# Autodesk Inventor assembly: MM3_3
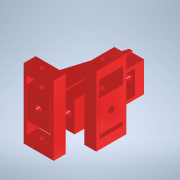
[picture p0: Inventor's stored thumbnail of the model, 180x180]
Saved by Autodesk Inventor 2021 (Build 250183000, 183)
## iProperties
Created: 2021-02-23
Part Number: MM3_3
Document SubType Name: Assembly
Designer: dsdan
Author: dsdan
## Documents named in this file (3)
- E:\OneDrive - Imperial College London\DragonVision_DanielKo\Instrumentation\Ephys_rig_2021\MM3_3.iam
- E:\OneDrive - Imperial College London\DragonVision_DanielKo\Instrumentation\Ephys_rig_2021\MM3.iam
- E:\OneDrive - Imperial College London\DragonVision_DanielKo\Instrumentation\Ephys_rig_2021\MM3_vertical.ipt
## Components (4 placed, 2 different names)
1. MM3:1 [sub-assembly] — Mate:1, Mate:2, Flush:1, Mate:4, Angle:1
2. MM3_vertical:1 — Mate:1, Mate:2, Flush:1, Mate:3, Flush:2
3. MM3:3 [sub-assembly] — Mate:3, Flush:2, Mate:4, Mate:5, Mate:6
4. MM3:4 [sub-assembly] — Mate:5, Angle:1, Mate:6
## Relationships (9: Mate 6, Flush 2, Angle 1)
- Mate:1: MM3:1 ↔ MM3_vertical:1
- Mate:2: MM3:1 ↔ MM3_vertical:1
- Flush:1: MM3:1 ↔ MM3_vertical:1
- Mate:3: MM3_vertical:1 ↔ MM3:3
- Flush:2: MM3_vertical:1 ↔ MM3:3
- Mate:4: MM3:1 ↔ MM3:3
- Mate:5: MM3:3 ↔ MM3:4
- Angle:1 (0 deg): MM3:1 ↔ MM3:4
- Mate:6: MM3:3 ↔ MM3:4
